# Autodesk Inventor assembly: BashyWingtip
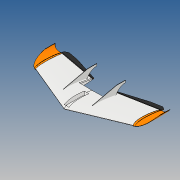
[picture p0: Inventor's stored thumbnail of the model, 180x180]
Saved by Autodesk Inventor 2019.4 (Build 234330000, 330)
## iProperties
Part Number: BashyWingtip
Document SubType Name: Assembly
Designer: Admin
Mass: 86342.2 g
Surface Area: 8991.76 cm^2
Volume: 10985 cm^3
Density: 7.86 g/cm^3
Revision: -
VAULT_Status: in Bearbeitung
Gewicht: 86,342 kg
InventorVersion: 2019.4
Author: Admin
## Documents named in this file (6)
- C:\Users\tonn\Documents\GitHub\CAD_Elements\CAD\bashy\BashyWingtip.iam
- BASHYWINGTIP_BASHYWINGTIP.IAM
- C:\Users\tonn\Documents\GitHub\CAD_Elements\CAD\bashy\Wingtip.ipt
- C:\Users\tonn\Documents\GitHub\CAD_Elements\CAD\bashy\Wing_airfoil.ipt
- C:\Users\tonn\Documents\GitHub\CAD_Elements\CAD\bashy\1X012705.ipt
- C:\Users\tonn\Documents\GitHub\CAD_Elements\CAD\bashy\Center_fin.ipt
## Components (5 placed, 4 different names)
1. WING_AIRFOIL_WINGTIP:1 — Fluchtend:1, Fluchtend:2, Passend:2, Passend:3, Fluchtend:3
2. WING_AIRFOIL_WING_AIRFOIL:1 — Fluchtend:1, Fluchtend:2, Passend:1, Passend:3, Fluchtend:4, Fluchtend:7
3. 1X012705_1X012705:1 — Passend:1, Passend:2, Fluchtend:3
4. CENTER_FIN_CENTER_FIN:1 — Fluchtend:5, Fluchtend:6
5. CENTER_FIN_CENTER_FIN:2 — Fluchtend:5, Fluchtend:6, Fluchtend:7
## Relationships (10: Flush 7, Mate 3)
- Fluchtend:1 [Flush]: WING_AIRFOIL_WINGTIP:1 ↔ WING_AIRFOIL_WING_AIRFOIL:1
- Fluchtend:2 [Flush]: WING_AIRFOIL_WINGTIP:1 ↔ WING_AIRFOIL_WING_AIRFOIL:1
- Passend:1 [Mate]: WING_AIRFOIL_WING_AIRFOIL:1 ↔ 1X012705_1X012705:1
- Passend:2 [Mate]: WING_AIRFOIL_WINGTIP:1 ↔ 1X012705_1X012705:1
- Passend:3 [Mate]: WING_AIRFOIL_WINGTIP:1 ↔ WING_AIRFOIL_WING_AIRFOIL:1
- Fluchtend:3 [Flush]: WING_AIRFOIL_WINGTIP:1 ↔ 1X012705_1X012705:1
- Fluchtend:4 [Flush] (-120 mm): WING_AIRFOIL_WING_AIRFOIL:1
- Fluchtend:5 [Flush]: CENTER_FIN_CENTER_FIN:1 ↔ CENTER_FIN_CENTER_FIN:2
- Fluchtend:6 [Flush]: CENTER_FIN_CENTER_FIN:1 ↔ CENTER_FIN_CENTER_FIN:2
- Fluchtend:7 [Flush] (120 mm): WING_AIRFOIL_WING_AIRFOIL:1 ↔ CENTER_FIN_CENTER_FIN:2
## Named parameters: Gewicht = 86.3422
note: some values were not read from the file. Shown as the stored number, unit unknown: "Gewicht".
